# Autodesk Inventor assembly: 01-gobeur-v3_asm
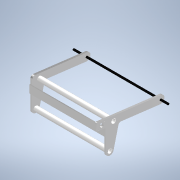
[picture p0: Inventor's stored thumbnail of the model, 180x180]
Saved by Autodesk Inventor 2020 (Build 240168000, 168)
## iProperties
Created: 2020-01-16
Part Number: 01-gobeur-v3_asm
Document SubType Name: Assembly
Designer: kwruff
Sending System: CREO PARAMETRIC BY PTC INC, 2019080
Preprocessor: CREO PARAMETRIC BY PTC INC, 2019080
Title: 01-GOBEUR-V3_ASM
Author: 1cikaychapman
Revision Number: 1LAST_VERSION
## Documents named in this file (6)
- \\CNOCMF05\Staff_R$\kwruff\My Documents\Downloads\folder to upload\01-gobeur-v3_asm.iam
- \\CNOCMF05\Staff_R$\kwruff\My Documents\Downloads\folder to upload\PLAQUECONNEXIONBRA0001.ipt
- \\CNOCMF05\Staff_R$\kwruff\My Documents\Downloads\folder to upload\GOBEUR_BRAS_V3.ipt
- \\CNOCMF05\Staff_R$\kwruff\My Documents\Downloads\folder to upload\GOBEUR_BRAS_MOTEUR_V3.ipt
- \\CNOCMF05\Staff_R$\kwruff\My Documents\Downloads\folder to upload\SHAFT05PO00.ipt
- \\CNOCMF05\Staff_R$\kwruff\My Documents\Downloads\folder to upload\PVC Roller.ipt
## Components (8 placed, 7 different names)
1. 0
2. 1
3. 2
4. 3 — Insert:1, Insert:2
5. 4
6. 5
7. PVC Roller:1 — Insert:2
8. PVC Roller:2 — Insert:1
## Relationships (2: Insert 2)
- Insert:1: 3 ↔ PVC Roller:2
- Insert:2: 3 ↔ PVC Roller:1
